# Autodesk Inventor assembly: DoublePulleyGearbox
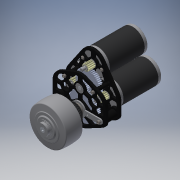
[picture p0: Inventor's stored thumbnail of the model, 180x180]
Saved by Autodesk Inventor 2016 (Build 200138000, 138)
## iProperties
Created: 2017-01-16
Part Number: DoublePulleyGearbox
Document SubType Name: Assembly
Designer: Kyle
Author: Kyle
## Documents named in this file (9)
- F:\FRC\2017\DriveTrainRev2\Individual Parts\DoublePulleyGearbox.iam
- F:\FRC\2017\DriveTrainRev2\Individual Parts\WCPSS.iam
- F:\FRC\2017\DriveTrainRev2\Individual Parts\.5Bearing.ipt
- F:\FRC\2017\DriveTrainRev2\Individual Parts\4x2Colson.ipt
- F:\FRC\2017\DriveTrainRev2\GearboxPlate.ipt
- F:\FRC\2017\DriveTrainRev2\Individual Parts\24t9MMPulley6mm.ipt
- F:\FRC\2017\DriveTrainRev2\Individual Parts\24t9MMPulleyExtension.ipt
- F:\FRC\2017\DriveTrainRev2\Individual Parts\.5HexBearing.ipt
- F:\FRC\2017\DriveTrainRev2\Individual Parts\.106Spacer.ipt
## Components (9 placed, 8 different names)
1. WCPSS:1 [sub-assembly] — Mate:1, Flush:1, Mate:2, Mate:4, Mate:5, Mate:6, Mate:12, Mate:14, Mate:15, Mate:16
2. .5Bearing:1 — Mate:1, Flush:1, Mate:3
3. 4x2Colson:1 — Mate:2, Mate:3, Mate:13
4. GearboxPlate:1 — Mate:4, Mate:5, Mate:6
5. 24t9MMPulley6mm:1 — Mate:7, Mate:8, Mate:9, Mate:10, Mate:13
6. 24t9MMPulley6mm:2 — Mate:10, Mate:11, Mate:12, Mate:17
7. 24t9MMPulleyExtension:1 — Mate:7, Mate:8, Mate:9, Mate:11
8. .5HexBearing:1 — Mate:14, Mate:15
9. .106Spacer:1 — Mate:16, Mate:17
## Relationships (18: Mate 17, Flush 1)
- Mate:1: WCPSS:1 ↔ .5Bearing:1
- Flush:1: WCPSS:1 ↔ .5Bearing:1
- Mate:2: WCPSS:1 ↔ 4x2Colson:1
- Mate:3: .5Bearing:1 ↔ 4x2Colson:1
- Mate:4: WCPSS:1 ↔ GearboxPlate:1
- Mate:5: WCPSS:1 ↔ GearboxPlate:1
- Mate:6: WCPSS:1 ↔ GearboxPlate:1
- Mate:7: 24t9MMPulley6mm:1 ↔ 24t9MMPulleyExtension:1
- Mate:8: 24t9MMPulley6mm:1 ↔ 24t9MMPulleyExtension:1
- Mate:9: 24t9MMPulley6mm:1 ↔ 24t9MMPulleyExtension:1
- Mate:10: 24t9MMPulley6mm:1 ↔ 24t9MMPulley6mm:2
- Mate:11: 24t9MMPulley6mm:2 ↔ 24t9MMPulleyExtension:1
- Mate:12: WCPSS:1 ↔ 24t9MMPulley6mm:2
- Mate:13: 4x2Colson:1 ↔ 24t9MMPulley6mm:1
- Mate:14: WCPSS:1 ↔ .5HexBearing:1
- Mate:15: WCPSS:1 ↔ .5HexBearing:1
- Mate:16: WCPSS:1 ↔ .106Spacer:1
- Mate:17: 24t9MMPulley6mm:2 ↔ .106Spacer:1
